# Autodesk Inventor assembly: component box all
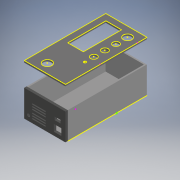
[picture p0: Inventor's stored thumbnail of the model, 180x180]
Saved by Autodesk Inventor 2021 (Build 250183000, 183)
## iProperties
Created: 2023-01-12
Part Number: component box all
Document SubType Name: Assembly
Designer: boyle
Author: boyle
## Documents named in this file (4)
- C:\Users\boyle\OneDrive\Documents\college\EExxx\EE420\NASA-Vestibular-Chair\Engineering Notebook\Brandon Boyle-Fagan\SD boxes\component box all.iam
- C:\Users\boyle\OneDrive\Documents\college\EExxx\EE420\NASA-Vestibular-Chair\Engineering Notebook\Brandon Boyle-Fagan\SD boxes\Component box Bottom.ipt
- C:\Users\boyle\OneDrive\Documents\college\EExxx\EE420\NASA-Vestibular-Chair\Engineering Notebook\Brandon Boyle-Fagan\SD boxes\component box cover.ipt
- C:\Users\boyle\OneDrive\Documents\college\EExxx\EE420\NASA-Vestibular-Chair\Engineering Notebook\Brandon Boyle-Fagan\SD boxes\compnent box front.ipt
## Components (3 placed, 3 different names)
1. Component box Bottom:1 — Mate:1, Flush:1, Flush:2
2. component box cover:1
3. compnent box front:1 — Mate:1, Flush:1, Flush:2
## Relationships (3: Flush 2, Mate 1)
- Mate:1: Component box Bottom:1 ↔ compnent box front:1
- Flush:1: Component box Bottom:1 ↔ compnent box front:1
- Flush:2: Component box Bottom:1 ↔ compnent box front:1
